# Autodesk Inventor assembly: Base Assembly 1
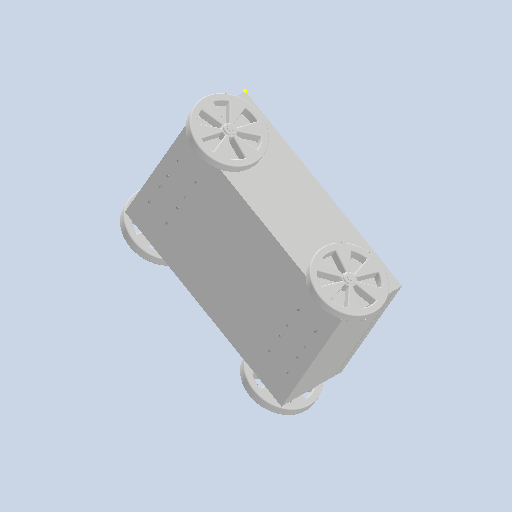
[picture p0: Inventor's stored thumbnail of the model, 512x512]
Saved by Autodesk Inventor 2022 (Build 260153000, 153)
## iProperties
Created: 2021-07-03
Part Number: Base Assembly 1
Document SubType Name: Assembly
Designer: parag
Author: parag
## Documents named in this file (8)
- F:\BVB\robotic arm\Base Assembly 1.iam
- F:\BVB\robotic arm\base.ipt
- F:\BVB\robotic arm\dc motor clamp.ipt
- F:\BVB\robotic arm\wheel shaft2.ipt
- F:\BVB\robotic arm\screw EE.ipt
- F:\BVB\robotic arm\wheel final.ipt
- F:\BVB\robotic arm\base cap.ipt
- F:\BVB\robotic arm\Grove_Ultrasonic_Sensor_V2.0.iam
## Components (37 placed, 7 different names)
1. base:1 — Mate:1, Mate:2, Mate:3, Mate:4, Mate:9, Mate:10, Mate:11, Mate:12, Mate:13, Mate:14, Mate:15, Mate:16, Mate:17, Mate:18, Mate:19, Mate:20, Mate:39, Mate:41, Mate:42, Mate:43, Mate:56, Flush:30, Flush:33, Flush:36, Mate:59, Flush:37, Flush:38
2. dc motor clamp:1 — Mate:9, Mate:10, Mate:19, Mate:33, Mate:35, Mate:36, Mate:37, Flush:13, Flush:14, Flush:15, Flush:16
3. dc motor clamp:2 — Mate:11, Mate:12, Mate:20, Mate:34, Mate:38, Mate:40, Flush:17, Flush:18, Flush:19, Flush:20
4. dc motor clamp:3 — Mate:13, Mate:14, Mate:18, Mate:29, Mate:30, Mate:31, Mate:32, Flush:9, Flush:10, Flush:11, Flush:12
5. dc motor clamp:4 — Mate:15, Mate:16, Mate:17, Mate:25, Flush:5, Mate:26, Mate:27, Mate:28, Flush:6, Flush:7, Flush:8
6. screw EE:1 — Mate:25, Flush:5
7. screw EE:2 — Mate:26, Flush:6
8. screw EE:3 — Mate:27, Flush:7
9. screw EE:4 — Mate:28, Flush:8
10. base cap:1 — Mate:41, Mate:42, Mate:43, Mate:44, Mate:45, Mate:46, Mate:47, Flush:21, Flush:22, Flush:23, Flush:24, Flush:29
11. wheel shaft2:5 — Mate:2, Mate:59, Flush:37, Rotational:5
12. wheel shaft2:6 — Mate:3, Mate:50, Rotational:4, Flush:36
13. wheel shaft2:7 — Mate:4, Mate:48, Rotational:1, Flush:33
14. wheel shaft2:8 — Mate:1, Flush:38, Rotational:6
15. screw EE:5 — Mate:32, Flush:11
16. screw EE:6 — Mate:35, Flush:15
17. screw EE:7 — Mate:34, Flush:18
18. screw EE:8 — Mate:36, Flush:14
19. screw EE:9 — Mate:40, Flush:17
20. screw EE:10 — Mate:47, Flush:22
21. screw EE:11 — Mate:39, Flush:20
22. screw EE:12 — Mate:38, Flush:19
23. screw EE:13 — Mate:33, Flush:13
24. screw EE:14 — Mate:29, Flush:9
25. screw EE:15 — Mate:30, Flush:10
26. screw EE:16 — Mate:31, Flush:12
27. screw EE:17 — Mate:37, Flush:16
28. screw EE:18 — Mate:44, Flush:21
29. screw EE:19 — Mate:45, Flush:24
30. screw EE:21 — Mate:46, Flush:23
31. wheel final:1 — Mate:50, Rotational:4
32. wheel final:2 — Rotational:6
33. wheel final:3 — Rotational:5
34. wheel final:4 — Mate:48, Rotational:1
35. Ultrasonic Ranger V2_0:1 [sub-assembly] — Mate:56, Flush:29, Flush:30, Mate:57, Mate:58, Flush:31, Flush:32
36. screw EE:22 — Mate:58, Flush:31
37. screw EE:23 — Mate:57, Flush:32
## Relationships (77: Mate 45, Flush 28, RevoluteJoint 4)
- Mate:1: base:1 ↔ wheel shaft2:8
- Mate:2: base:1 ↔ wheel shaft2:5
- Mate:3: base:1 ↔ wheel shaft2:6
- Mate:4: base:1 ↔ wheel shaft2:7
- Mate:9: base:1 ↔ dc motor clamp:1
- Mate:10: base:1 ↔ dc motor clamp:1
- Mate:11: base:1 ↔ dc motor clamp:2
- Mate:12: base:1 ↔ dc motor clamp:2
- Mate:13: base:1 ↔ dc motor clamp:3
- Mate:14: base:1 ↔ dc motor clamp:3
- Mate:15: base:1 ↔ dc motor clamp:4
- Mate:16: base:1 ↔ dc motor clamp:4
- Mate:17 (34 mm): base:1 ↔ dc motor clamp:4
- Mate:18 (34 mm): base:1 ↔ dc motor clamp:3
- Mate:19 (34 mm): base:1 ↔ dc motor clamp:1
- Mate:20 (34 mm): base:1 ↔ dc motor clamp:2
- Mate:25: dc motor clamp:4 ↔ screw EE:1
- Flush:5 (-2.4 mm): dc motor clamp:4 ↔ screw EE:1
- Mate:26: dc motor clamp:4 ↔ screw EE:2
- Mate:27: dc motor clamp:4 ↔ screw EE:3
- Mate:28: dc motor clamp:4 ↔ screw EE:4
- Mate:29: dc motor clamp:3 ↔ screw EE:14
- Mate:30: dc motor clamp:3 ↔ screw EE:15
- Mate:31: dc motor clamp:3 ↔ screw EE:16
- Mate:32: dc motor clamp:3 ↔ screw EE:5
- Mate:33: dc motor clamp:1 ↔ screw EE:13
- Mate:34: dc motor clamp:2 ↔ screw EE:7
- Mate:35: dc motor clamp:1 ↔ screw EE:6
- Mate:36: dc motor clamp:1 ↔ screw EE:8
- Mate:37: dc motor clamp:1 ↔ screw EE:17
- Mate:38: dc motor clamp:2 ↔ screw EE:12
- Mate:39: base:1 ↔ screw EE:11
- Mate:40: dc motor clamp:2 ↔ screw EE:9
- Flush:6 (-2.4 mm): dc motor clamp:4 ↔ screw EE:2
- Flush:7 (2.4 mm): dc motor clamp:4 ↔ screw EE:3
- Flush:8 (2.4 mm): dc motor clamp:4 ↔ screw EE:4
- Flush:9 (2.4 mm): dc motor clamp:3 ↔ screw EE:14
- Flush:10 (2.4 mm): dc motor clamp:3 ↔ screw EE:15
- Flush:11 (2.4 mm): dc motor clamp:3 ↔ screw EE:5
- Flush:12 (2.4 mm): dc motor clamp:3 ↔ screw EE:16
- Flush:13 (2.4 mm): dc motor clamp:1 ↔ screw EE:13
- Flush:14 (2.4 mm): dc motor clamp:1 ↔ screw EE:8
- Flush:15 (2.4 mm): dc motor clamp:1 ↔ screw EE:6
- Flush:16 (2.4 mm): dc motor clamp:1 ↔ screw EE:17
- Flush:17 (2.4 mm): dc motor clamp:2 ↔ screw EE:9
- Flush:18 (2.4 mm): dc motor clamp:2 ↔ screw EE:7
- Flush:19 (2.4 mm): dc motor clamp:2 ↔ screw EE:12
- Flush:20 (2.4 mm): dc motor clamp:2 ↔ screw EE:11
- Mate:41: base:1 ↔ base cap:1
- Mate:42: base:1 ↔ base cap:1
- Mate:43: base:1 ↔ base cap:1
- Mate:44: base cap:1 ↔ screw EE:18
- Mate:45: base cap:1 ↔ screw EE:19
- Mate:46: base cap:1 ↔ screw EE:21
- Mate:47: base cap:1 ↔ screw EE:10
- Flush:21 (2.4 mm): base cap:1 ↔ screw EE:18
- Flush:22 (2.4 mm): base cap:1 ↔ screw EE:10
- Flush:23 (-2.4 mm): base cap:1 ↔ screw EE:21
- Flush:24 (2.4 mm): base cap:1 ↔ screw EE:19
- Mate:48: wheel shaft2:7 ↔ wheel final:4
- Mate:50: wheel shaft2:6 ↔ wheel final:1
- Mate:56: base:1 ↔ Ultrasonic Ranger V2_0:1
- Flush:29 (-27 mm): base cap:1 ↔ Ultrasonic Ranger V2_0:1
- Flush:30 (-75 mm): base:1 ↔ Ultrasonic Ranger V2_0:1
- Mate:57: Ultrasonic Ranger V2_0:1 ↔ screw EE:23
- Mate:58: Ultrasonic Ranger V2_0:1 ↔ screw EE:22
- Flush:31 (-3 mm): Ultrasonic Ranger V2_0:1 ↔ screw EE:22
- Flush:32 (3 mm): Ultrasonic Ranger V2_0:1 ↔ screw EE:23
- Rotational:1 [RevoluteJoint] (-1 mm): wheel shaft2:7 ↔ wheel final:4
- Flush:33 (20 mm): base:1 ↔ wheel shaft2:7
- Rotational:4 [RevoluteJoint] (-1 mm): wheel shaft2:6 ↔ wheel final:1
- Flush:36 (20 mm): base:1 ↔ wheel shaft2:6
- Mate:59: base:1 ↔ wheel shaft2:5
- Flush:37 (20 mm): base:1 ↔ wheel shaft2:5
- Flush:38 (20 mm): base:1 ↔ wheel shaft2:8
- Rotational:5 [RevoluteJoint] (-1 mm): wheel shaft2:5 ↔ wheel final:3
- Rotational:6 [RevoluteJoint] (-1 mm): wheel shaft2:8 ↔ wheel final:2
